# Autodesk Inventor assembly: LowerBody_MIR
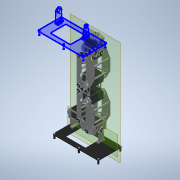
[picture p0: Inventor's stored thumbnail of the model, 180x180]
Saved by Autodesk Inventor 2020 (Build 240168000, 168)
## iProperties
Created: 2021-10-01
Part Number: LowerBody_MIR
Document SubType Name: Assembly
Designer: Masato Kubotera
Mass: 1009.03 g
Surface Area: 2721.67 cm^2
Volume: 456.516 cm^3
Density: 2.21029 g/cm^3
Author: Masato
## Documents named in this file (13)
- C:\Users\Masato\Documents\Inventor\CIT Brains_Inventor\OpenPlatform_ver3_0\LowerBody\LowerBody_MIR.iam
- C:\Users\Masato\Documents\Inventor\CIT Brains_Inventor\OpenPlatform_ver3_0\LowerBody\Ankle\Ankle.iam
- C:\Users\Masato\Documents\Inventor\CIT Brains_Inventor\OpenPlatform_ver3_0\LowerBody\Ankle\Ankle_side_pitch.iam
- C:\Users\Masato\Documents\Inventor\CIT Brains_Inventor\OpenPlatform_ver3_0\LowerBody\Knee\Knee.iam
- C:\Users\Masato\Documents\Inventor\CIT Brains_Inventor\OpenPlatform_ver3_0\LowerBody\Leg_joit\Leg_joint_roll_pitch.iam
- C:\Users\Masato\Documents\Inventor\CIT Brains_Inventor\OpenPlatform_ver3_0\LowerBody\Leg_joit\Leg_joint_roll_yaw.iam
- C:\Users\Masato\Documents\Inventor\CIT Brains_Inventor\OpenPlatform_ver3_0\LowerBody\Slider_crank\Slider_crank_mechanism.iam
- C:\Users\Masato\Documents\Inventor\CIT Brains_Inventor\OpenPlatform_ver3_0\LowerBody\Link\BackLink.iam
- C:\Users\Masato\Documents\Inventor\CIT Brains_Inventor\OpenPlatform_ver3_0\LowerBody\Link\FrontLink.iam
- C:\Users\Masato\Documents\Inventor\CIT Brains_Inventor\OpenPlatform_ver3_0\Ready_Made\Screw\M2_6-6.ipt
- C:\Users\Masato\Documents\Inventor\CIT Brains_Inventor\OpenPlatform_ver3_0\Ready_Made\Screw\M3-6.ipt
- C:\Users\Masato\Documents\Inventor\CIT Brains_Inventor\OpenPlatform_ver3_0\Ready_Made\Screw\M3-8.ipt
- C:\Users\Masato\Documents\Inventor\CIT Brains_Inventor\OpenPlatform_ver3_0\LowerBody\Foot\Foot_MIR.iam
## Components (36 placed, 12 different names)
1. Ankle:1 [sub-assembly] — 挿入:21, 挿入:22, 角度:11, 挿入:55
2. Ankle_side_pitch:1 [sub-assembly] — 挿入:21, フラッシュ:5, 挿入:36, 挿入:35, 挿入:23, 挿入:24, 挿入:25, 挿入:26
3. Ankle_side_pitch:2 [sub-assembly] — フラッシュ:5, 挿入:22, 挿入:27, 挿入:28, 挿入:29, 挿入:30
4. Knee:1 [sub-assembly] — 挿入:33, 挿入:31, 挿入:34, 挿入:32
5. Leg_joint_roll_pitch:1 [sub-assembly] — 挿入:70, 角度:6, 挿入:2, 挿入:38, 角度:9, 角度:10, 挿入:37
6. Leg_joint_roll_yaw:1 [sub-assembly] — 挿入:70, 角度:6, フラッシュ:4, フラッシュ:3, メイト:1, 挿入:69, 角度:10
7. Slider_crank_mechanism:1 [sub-assembly] — 挿入:69, 挿入:2
8. BackLink:1 [sub-assembly] — 挿入:36, 挿入:33, 角度:7, 挿入:42, 挿入:46, 挿入:64, 挿入:66
9. FrontLink:1 [sub-assembly] — 角度:11, 角度:7, 挿入:35, 挿入:31, 角度:12, 挿入:63, 挿入:65
10. BackLink:2 [sub-assembly] — 挿入:34, 挿入:38, 角度:8, 挿入:39, 挿入:44, 挿入:41, 挿入:45
11. FrontLink:2 [sub-assembly] — 角度:9, 角度:12, 角度:10, 角度:8, 挿入:32, 挿入:37, 挿入:40, 挿入:43
12. M2_6-6:1
13. M2_6-6:2
14. M2_6-6:3
15. M2_6-6:4
16. M2_6-6:5 — 挿入:23
17. M2_6-6:6 — 挿入:24
18. M2_6-6:7 — 挿入:25
19. M2_6-6:8 — 挿入:26
20. M2_6-6:9 — 挿入:27
21. M2_6-6:10 — 挿入:28
22. M2_6-6:11 — 挿入:29
23. M2_6-6:12 — 挿入:30
24. M3-6:1 — 挿入:40
25. M3-6:2 — 挿入:39
26. M3-6:3 — 挿入:44
27. M3-6:4 — 挿入:43
28. M3-6:5 — 挿入:41
29. M3-6:6 — 挿入:45
30. M3-6:7 — 挿入:42
31. M3-6:8 — 挿入:46
32. M3-8:1 — 挿入:63
33. M3-8:2 — 挿入:64
34. M3-8:3 — 挿入:66
35. M3-8:4 — 挿入:65
36. Foot_MIR:1 [sub-assembly] — 挿入:55, 角度:10
## Relationships (46: Insert 34, Angle 8, Flush 2, Mate 2)
- 挿入:21 [Insert]: Ankle:1 ↔ Ankle_side_pitch:1
- フラッシュ:5 [Flush]: Ankle_side_pitch:1 ↔ Ankle_side_pitch:2
- 挿入:22 [Insert]: Ankle:1 ↔ Ankle_side_pitch:2
- 挿入:70 [Insert]: Leg_joint_roll_pitch:1 ↔ Leg_joint_roll_yaw:1
- 角度:6 [Angle] (0 deg): Leg_joint_roll_pitch:1 ↔ Leg_joint_roll_yaw:1
- フラッシュ:4 [Mate]: Leg_joint_roll_yaw:1
- フラッシュ:3 [Flush]: Leg_joint_roll_yaw:1
- メイト:1 [Mate]: Leg_joint_roll_yaw:1
- 挿入:69 [Insert]: Leg_joint_roll_yaw:1 ↔ Slider_crank_mechanism:1
- 挿入:2 [Insert]: Leg_joint_roll_pitch:1 ↔ Slider_crank_mechanism:1
- 挿入:36 [Insert]: Ankle_side_pitch:1 ↔ BackLink:1
- 挿入:33 [Insert]: Knee:1 ↔ BackLink:1
- 角度:11 [Angle] (0 deg): Ankle:1 ↔ FrontLink:1
- 角度:7 [Angle] (0 deg): BackLink:1 ↔ FrontLink:1
- 挿入:35 [Insert]: Ankle_side_pitch:1 ↔ FrontLink:1
- 挿入:31 [Insert]: Knee:1 ↔ FrontLink:1
- 挿入:34 [Insert]: Knee:1 ↔ BackLink:2
- 挿入:38 [Insert]: Leg_joint_roll_pitch:1 ↔ BackLink:2
- 角度:9 [Angle] (0 deg): Leg_joint_roll_pitch:1 ↔ FrontLink:2
- 角度:12 [Angle] (0 deg): FrontLink:1 ↔ FrontLink:2
- 角度:10 [Angle] (0 deg): Leg_joint_roll_pitch:1 ↔ FrontLink:2
- 角度:8 [Angle] (0 deg): BackLink:2 ↔ FrontLink:2
- 挿入:32 [Insert]: Knee:1 ↔ FrontLink:2
- 挿入:37 [Insert]: Leg_joint_roll_pitch:1 ↔ FrontLink:2
- 挿入:23 [Insert]: Ankle_side_pitch:1 ↔ M2_6-6:5
- 挿入:24 [Insert]: Ankle_side_pitch:1 ↔ M2_6-6:6
- 挿入:25 [Insert]: Ankle_side_pitch:1 ↔ M2_6-6:7
- 挿入:26 [Insert]: Ankle_side_pitch:1 ↔ M2_6-6:8
- 挿入:27 [Insert]: Ankle_side_pitch:2 ↔ M2_6-6:9
- 挿入:28 [Insert]: Ankle_side_pitch:2 ↔ M2_6-6:10
- 挿入:29 [Insert]: Ankle_side_pitch:2 ↔ M2_6-6:11
- 挿入:30 [Insert]: Ankle_side_pitch:2 ↔ M2_6-6:12
- 挿入:40 [Insert]: FrontLink:2 ↔ M3-6:1
- 挿入:39 [Insert]: BackLink:2 ↔ M3-6:2
- 挿入:44 [Insert]: BackLink:2 ↔ M3-6:3
- 挿入:43 [Insert]: FrontLink:2 ↔ M3-6:4
- 挿入:41 [Insert]: BackLink:2 ↔ M3-6:5
- 挿入:45 [Insert]: BackLink:2 ↔ M3-6:6
- 挿入:42 [Insert]: BackLink:1 ↔ M3-6:7
- 挿入:46 [Insert]: BackLink:1 ↔ M3-6:8
- 挿入:63 [Insert]: FrontLink:1 ↔ M3-8:1
- 挿入:64 [Insert]: BackLink:1 ↔ M3-8:2
- 挿入:66 [Insert]: BackLink:1 ↔ M3-8:3
- 挿入:65 [Insert]: FrontLink:1 ↔ M3-8:4
- 挿入:55 [Insert]: Ankle:1 ↔ Foot_MIR:1
- 角度:10 [Angle] (0 deg): Leg_joint_roll_yaw:1 ↔ Foot_MIR:1
